# Autodesk Inventor assembly: 6P Sprocket
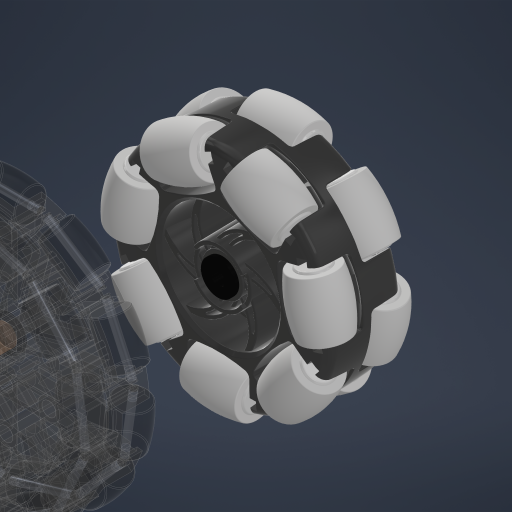
[picture p0: Inventor's stored thumbnail of the model, 512x512]
Saved by Autodesk Inventor 2023.2 (Build 272271000, 271)
## iProperties
Created: 2022-08-02
Part Number: 6P Sprocket
Document SubType Name: Assembly
Designer: ylu12
Author: ylu12
## Documents named in this file (4)
- D:\CAD\Parts\standard\Motion\Wheels\Omni Wheels\Omni Wheel\2.75 Omni, Circle.iam
- D:\CAD\Parts\standard\Motion\Wheels\Omni Wheels\Reference Parts\2.75 Omni.ipt
- D:\CAD\Parts\standard\Motion\Adapters\Insert Circle.ipt
- D:\CAD\Parts\standard\Motion\Wheels\Omni Wheels\Omni Wheel.iam
## Components (3 placed, 3 different names)
1. 2.75 Omni
2. Circle 1 — Flush:12, Flush:13, Flush:14, Mate:20, Angle:2
3. Circle 2 — Flush:12, Flush:13, Mate:19
## Relationships (9: Mate 4, Flush 4, Angle 1)
- [Mate]: 2.75 Omni
- [Mate]: 2.75 Omni
- [Flush]: 2.75 Omni
- Flush:12: Circle 1 ↔ Circle 2
- Flush:13: Circle 1 ↔ Circle 2
- Mate:19 (9.98 mm): Circle 2
- Flush:14 (9.98 mm): Circle 1
- Mate:20: Circle 1
- Angle:2 (0 deg): Circle 1
## Named parameters: HalfWheelWidth = 9.98 mm
